# Autodesk Inventor assembly: 2018 sidepontoon booled assen
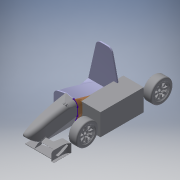
[picture p0: Inventor's stored thumbnail of the model, 180x180]
Saved by Autodesk Inventor 2018 (Build 220112000, 112)
## iProperties
Company: none
Created: 2018-02-15
Part Number: 2018 sidepontoon booled assen
Material: 一般
Description: CATIA V5 STEP Exchange
Document SubType Name: Assembly
Designer: kit
Authority: none
Sending System: CATIA V5 STEP AP203
Preprocessor: CATIA Version 5 Release 17 (IN-10)
Title: Z:\各班フォルダ\2018\ボディ\カウル\AeroCAD2018\CAD\stl\2018 radiator analysis1.stp
Author: none
## Documents named in this file (10)
- C:\Users\kit\Documents\Inventor\aero cad\新しいフォルダー\AeroCAD2018\CAD\Inventor\Aero Parts\Side Pontoon\2018 sidepontoon booled assen.iam
- C:\Users\kit\Documents\Inventor\aero cad\新しいフォルダー\AeroCAD2018\CAD\stl\radiator_analysisradiator 2018.ipt
- C:\Users\kit\Documents\Inventor\aero cad\新しいフォルダー\AeroCAD2018\CAD\stl\radiator_analysisAssyTsutsui2018.iam
- C:\Users\kit\Documents\Inventor\aero cad\新しいフォルダー\AeroCAD2018\CAD\stl\radiator_analysisPart123.ipt
- C:\Users\kit\Documents\Inventor\aero cad\新しいフォルダー\AeroCAD2018\CAD\stl\radiator_analysisSidePanel_Upper.ipt
- C:\Users\kit\Documents\Inventor\aero cad\新しいフォルダー\AeroCAD2018\CAD\stl\radiator_analysisPart132.1.ipt
- C:\Users\kit\Documents\Inventor\aero cad\新しいフォルダー\AeroCAD2018\CAD\stl\radiator_analysisF-wing.iam
- C:\Users\kit\Documents\Inventor\aero cad\新しいフォルダー\AeroCAD2018\CAD\stl\radiator_analysisunderpanel middle.ipt
- C:\Users\kit\Documents\Inventor\aero cad\新しいフォルダー\AeroCAD2018\CAD\Inventor\Assembly(KS-14.ver)\2018 flame\LowBody.ipt
- C:\Users\kit\Documents\Inventor\aero cad\新しいフォルダー\AeroCAD2018\CAD\Inventor\Aero Parts\Side Pontoon\Side pontoon2.ipt
## Components (9 placed, 9 different names)
1. radiator 2018.1
2. AssyTsutsui2018.1 [sub-assembly]
3. sidepontoon.1
4. Part127.1
5. 2018Frontnose
6. F-wing.1 [sub-assembly]
7. underpanel middle.1
8. LowBody:1 — メイト:1
9. Side pontoon2:1 — メイト:2, メイト:3
## Relationships (3: Mate 3)
- メイト:1 [Mate]: LowBody:1
- メイト:2 [Mate]: Side pontoon2:1
- メイト:3 [Mate]: Side pontoon2:1
